# Autodesk Inventor assembly: viperx_hand
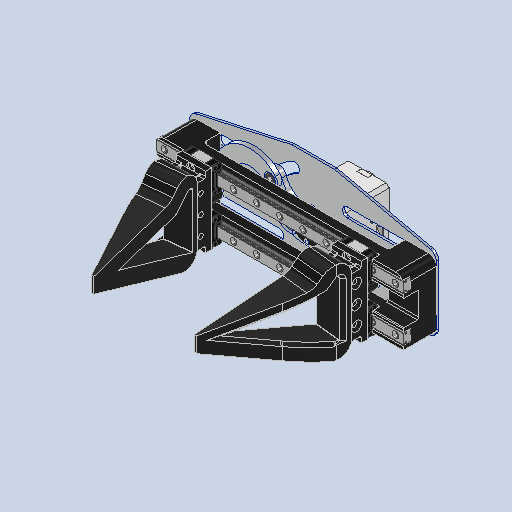
[picture p0: Inventor's stored thumbnail of the model, 512x512]
Saved by Autodesk Inventor 2024.3 (Build 283343010, 343A)
## iProperties
Created: 2025-06-26
Part Number: viperx_hand
Document SubType Name: Assembly
Designer: kshau
Author: kshau
## Documents named in this file (12)
- C:\Users\kshau\Documents\inventor\Create_ViperX\Create_ViperX_ALOHA\ViperX_hand\viperx_hand.iam
- C:\Users\kshau\Documents\inventor\Create_ViperX\Create_ViperX_ALOHA\ViperX_hand\bridge_rails_support.ipt
- C:\Users\kshau\Documents\inventor\Create_ViperX\Create_ViperX_ALOHA\ViperX_hand\finger_adaptor.ipt
- C:\Users\kshau\Documents\inventor\Create_ViperX\Create_ViperX_ALOHA\ViperX_hand\rotor.ipt
- C:\Users\kshau\Documents\inventor\Create_ViperX\Create_ViperX_ALOHA\ViperX_hand\rotor_arm.ipt
- C:\Users\kshau\Documents\inventor\Create_ViperX\Create_ViperX_ALOHA\NessesaryParts\NTN_WA673SA\WA673SA\WA673SA\WA673SA.ipt
- C:\Users\kshau\Documents\inventor\Create_ViperX\Create_ViperX_ALOHA\NessesaryParts\SSE2BSZ8-160_STEP_AP203_20250628\SSE2BSZ8-160\SSE2BSZ8-160\SSE2BSZ8-160.iam
- C:\Users\kshau\Documents\inventor\Create_ViperX\Create_ViperX_ALOHA\Actuator\XM,H-430_idler\XM,H-430_idler\XM,H-430_idler.iam
- C:\Users\kshau\Documents\inventor\Create_ViperX\Create_ViperX_ALOHA\ViperX_hand\joint_adaptor_plate.ipt
- C:\Users\kshau\Documents\inventor\Create_ViperX\Create_ViperX_ALOHA\ViperX_hand\rotor_shim.ipt
- C:\Users\kshau\Documents\inventor\Create_ViperX\Create_ViperX_ALOHA\ViperX_hand\finger.ipt
- C:\Users\kshau\Documents\inventor\Create_ViperX\Create_ViperX_ALOHA\ViperX_hand\finger_MIR1.ipt
## Components (19 placed, 11 different names)
1. bridge_rails_support:1 — 回転:5, 回転:6, 回転:7, 回転:8, 回転:15, 回転:16
2. finger_adaptor:1 — 回転:3, フラッシュ:1, 回転:9, 回転:10, メイト:15, メイト:16, メイト:17
3. rotor:1 — 回転:13, 回転:14, メイト:14
4. rotor_arm:1 — メイト:1, メイト:2, メイト:5, メイト:6, メイト:8, 回転:13
5. rotor_arm:2 — メイト:3, メイト:4, メイト:9, メイト:10, メイト:12, 回転:14
6. WA673SA:1 — メイト:1, メイト:2
7. WA673SA:2 — メイト:3, メイト:4
8. WA673SA:3 — メイト:5, メイト:6, メイト:7
9. WA673SA:4 — メイト:7, メイト:8, 回転:3
10. WA673SA:6 — メイト:11, メイト:12, 回転:4
11. WA673SA:7 — メイト:9, メイト:10, メイト:11
12. finger_adaptor:2 — 回転:4, フラッシュ:1, 回転:11, 回転:12, メイト:18, メイト:19, メイト:20
13. SSE2BSZ8-160:1 [sub-assembly] — 回転:5, 回転:6, 回転:10, 回転:11
14. SSE2BSZ8-160:2 [sub-assembly] — 回転:7, 回転:8, 回転:9, 回転:12
15. XM,H-430_idler:1 [sub-assembly] — メイト:14, 回転:17, 回転:18, 回転:19, 回転:20
16. joint_adaptor_plate:1 — 回転:15, 回転:16, 回転:17, 回転:18
17. rotor_shim:1 — 回転:19, 回転:20
18. finger:1 — メイト:15, メイト:16, メイト:17
19. finger_MIR1:1 — メイト:18, メイト:19, メイト:20
## Relationships (38: Mate 19, RevoluteJoint 18, Flush 1)
- メイト:1 [Mate]: rotor_arm:1 ↔ WA673SA:1
- メイト:2 [Mate]: rotor_arm:1 ↔ WA673SA:1
- メイト:3 [Mate]: rotor_arm:2 ↔ WA673SA:2
- メイト:4 [Mate]: rotor_arm:2 ↔ WA673SA:2
- メイト:5 [Mate]: rotor_arm:1 ↔ WA673SA:3
- メイト:6 [Mate]: rotor_arm:1 ↔ WA673SA:3
- メイト:7 [Mate]: WA673SA:3 ↔ WA673SA:4
- メイト:8 [Mate]: rotor_arm:1 ↔ WA673SA:4
- メイト:9 [Mate]: rotor_arm:2 ↔ WA673SA:7
- メイト:10 [Mate]: rotor_arm:2 ↔ WA673SA:7
- メイト:11 [Mate]: WA673SA:6 ↔ WA673SA:7
- メイト:12 [Mate]: rotor_arm:2 ↔ WA673SA:6
- 回転:3 [RevoluteJoint]: finger_adaptor:1 ↔ WA673SA:4
- 回転:4 [RevoluteJoint]: WA673SA:6 ↔ finger_adaptor:2
- フラッシュ:1 [Flush]: finger_adaptor:1 ↔ finger_adaptor:2
- 回転:5 [RevoluteJoint]: bridge_rails_support:1 ↔ SSE2BSZ8-160:1
- 回転:6 [RevoluteJoint]: bridge_rails_support:1 ↔ SSE2BSZ8-160:1
- 回転:7 [RevoluteJoint]: bridge_rails_support:1 ↔ SSE2BSZ8-160:2
- 回転:8 [RevoluteJoint]: bridge_rails_support:1 ↔ SSE2BSZ8-160:2
- 回転:9 [RevoluteJoint]: finger_adaptor:1 ↔ SSE2BSZ8-160:2
- 回転:10 [RevoluteJoint]: finger_adaptor:1 ↔ SSE2BSZ8-160:1
- 回転:11 [RevoluteJoint]: finger_adaptor:2 ↔ SSE2BSZ8-160:1
- 回転:12 [RevoluteJoint]: finger_adaptor:2 ↔ SSE2BSZ8-160:2
- 回転:13 [RevoluteJoint]: rotor:1 ↔ rotor_arm:1
- 回転:14 [RevoluteJoint]: rotor:1 ↔ rotor_arm:2
- メイト:14 [Mate]: rotor:1 ↔ XM,H-430_idler:1
- 回転:15 [RevoluteJoint]: bridge_rails_support:1 ↔ joint_adaptor_plate:1
- 回転:16 [RevoluteJoint]: bridge_rails_support:1 ↔ joint_adaptor_plate:1
- 回転:17 [RevoluteJoint]: XM,H-430_idler:1 ↔ joint_adaptor_plate:1
- 回転:18 [RevoluteJoint]: XM,H-430_idler:1 ↔ joint_adaptor_plate:1
- 回転:19 [RevoluteJoint]: XM,H-430_idler:1 ↔ rotor_shim:1
- 回転:20 [RevoluteJoint]: XM,H-430_idler:1 ↔ rotor_shim:1
- メイト:15 [Mate]: finger_adaptor:1 ↔ finger:1
- メイト:16 [Mate]: finger_adaptor:1 ↔ finger:1
- メイト:17 [Mate]: finger_adaptor:1 ↔ finger:1
- メイト:18 [Mate]: finger_adaptor:2 ↔ finger_MIR1:1
- メイト:19 [Mate]: finger_adaptor:2 ↔ finger_MIR1:1
- メイト:20 [Mate]: finger_adaptor:2 ↔ finger_MIR1:1
